# Autodesk Inventor assembly: ball_collector_assembly
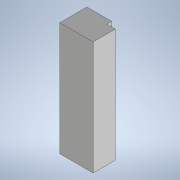
[picture p0: Inventor's stored thumbnail of the model, 180x180]
Saved by Autodesk Inventor 2020 (Build 240168000, 168)
## iProperties
Created: 2021-03-06
Part Number: ball_collector_assembly
Document SubType Name: Assembly
Designer: Harry
Author: Harry
## Documents named in this file (3)
- C:\Users\Harry\Documents\hacktheburgh\octocatch\cad\ball_collector_assembly.iam
- C:\Users\Harry\Documents\hacktheburgh\octocatch\cad\ball collector.ipt
- C:\Users\Harry\Documents\hacktheburgh\octocatch\cad\Sensor Ultrasonic.ipt
## Components (2 placed, 2 different names)
1. ball collector:1 — Insert:1
2. Sensor Ultrasonic:1 — Insert:1
## Relationships (1: Insert 1)
- Insert:1: ball collector:1 ↔ Sensor Ultrasonic:1
